# Autodesk Inventor assembly: module_switch
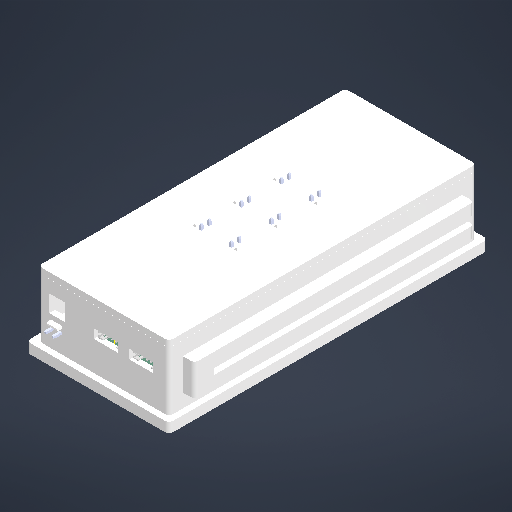
[picture p0: Inventor's stored thumbnail of the model, 512x512]
Saved by Autodesk Inventor 2025.2 (Build 292293000, 293)
## iProperties
Created: 2025-11-12
Part Number: module_switch
Document SubType Name: Assembly
Designer: sam
Author: sam
## Documents named in this file (4)
- G:\projects\primary\regulated-irrigation-system\model\asm\module-switch\module_switch.iam
- G:\projects\primary\regulated-irrigation-system\model\asm\module-switch\module_switch.ipt
- G:\projects\primary\regulated-irrigation-system\model\asm\module-switch\module-lid_switch.ipt
- G:\projects\primary\regulated-irrigation-system\model\asm\electronic-components\pcb_switch-module.iam
## Components (3 placed, 3 different names)
1. module_switch:1 — Mate:1, Mate:2, Mate:3, Mate:4, Mate:5
2. module-lid_switch:1 — Mate:1, Mate:2
3. pcb_switch-module:1 [sub-assembly] — Mate:3, Mate:4, Mate:5
## Relationships (5: Mate 5)
- Mate:1: module_switch:1 ↔ module-lid_switch:1
- Mate:2: module_switch:1 ↔ module-lid_switch:1
- Mate:3: module_switch:1 ↔ pcb_switch-module:1
- Mate:4 (0.2 mm): module_switch:1 ↔ pcb_switch-module:1
- Mate:5 (0.2 mm): module_switch:1 ↔ pcb_switch-module:1
